# Autodesk Inventor assembly: czlon 1 i 2
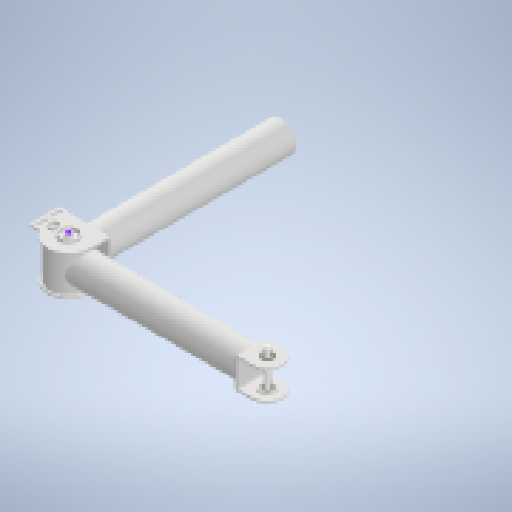
[picture p0: Inventor's stored thumbnail of the model, 512x512]
Saved by Autodesk Inventor 2023 (Build 270158000, 158)
## iProperties
Created: 2023-04-09
Part Number: czlon 1 i 2
Document SubType Name: Assembly
Designer: Wiktor
Author: Wiktor
## Documents named in this file (9)
- C:\Users\krzys\Documents\GitHub\Manipulator-Inventor\czlon 1 i 2.iam
- C:\Users\krzys\Documents\GitHub\Manipulator-Inventor\czlon i przekladnia.iam
- C:\Users\krzys\Documents\GitHub\Manipulator-Inventor\czlon 1 i 2\Design Accelerator\Łożysko1.iam
- C:\Users\krzys\Documents\GitHub\Manipulator-Inventor\Wał1.ipt
- C:\Users\krzys\Documents\GitHub\Manipulator-Inventor\czlon 1 i 2\Design Accelerator\Przekładnie walcowe1.iam
- C:\Users\krzys\Documents\GitHub\Manipulator-Inventor\czlon 1 i 2\Design Accelerator\Połączenie wpustowe1.iam
- C:\Users\krzys\Documents\GitHub\Manipulator-Inventor\czlon 2.ipt
- C:\Users\krzys\Documents\GitHub\Manipulator-Inventor\czlon 1 i 2\Design Accelerator\Łożysko2.iam
- C:\Users\krzys\Documents\GitHub\Manipulator-Inventor\Wał3.ipt
## Components (10 placed, 6 different names)
1. czlon i przekladnia:1 [sub-assembly] — Zestawiające:1, Zestawiające:2, Zestawiające:3, Zestawiające:4, Zestawiające:5, Kątowe:1, Równoległe:1
2. Łożysko:1 [sub-assembly] — Zestawiające:1, Zestawiające:2, Zestawiające:6, Zestawiające:7
3. Łożysko:3 [sub-assembly] — Zestawiające:3, Zestawiające:4, Zestawiające:5
4. Wał:1 — Zestawiające:6, Zestawiające:7, Kątowe:1, Zestawiające:10, Wstawiające:1
5. Przekładnie walcowe:1 [sub-assembly] — Wstawiające:1
6. Połączenie wpustowe:1 [sub-assembly]
7. czlon 2:1 — Zestawiające:10, Równoległe:1, Wstawiające:2, Wstawiające:3
8. Łożysko:4 [sub-assembly] — Wstawiające:3, Zestawiające:11, Równoległe:2, Kątowe:2
9. Łożysko:5 [sub-assembly] — Wstawiające:2
10. Wał:1 — Zestawiające:11, Równoległe:2, Kątowe:2
## Relationships (16: Mate 9, Insert 3, Angle 2, Flush 2)
- Zestawiające:1 [Mate]: czlon i przekladnia:1 ↔ Łożysko:1
- Zestawiające:2 [Mate]: czlon i przekladnia:1 ↔ Łożysko:1
- Zestawiające:3 [Mate]: czlon i przekladnia:1 ↔ Łożysko:3
- Zestawiające:4 [Mate]: czlon i przekladnia:1 ↔ Łożysko:3
- Zestawiające:5 [Mate]: czlon i przekladnia:1 ↔ Łożysko:3
- Zestawiające:6 [Mate]: Łożysko:1 ↔ Wał:1
- Zestawiające:7 [Mate]: Łożysko:1 ↔ Wał:1
- Kątowe:1 [Angle] (0 deg): czlon i przekladnia:1 ↔ Wał:1
- Zestawiające:10 [Mate]: Wał:1 ↔ czlon 2:1
- Równoległe:1 [Flush]: czlon i przekladnia:1 ↔ czlon 2:1
- Wstawiające:1 [Insert] (-20 mm): Wał:1 ↔ Przekładnie walcowe:1
- Wstawiające:2 [Insert]: czlon 2:1 ↔ Łożysko:5
- Wstawiające:3 [Insert]: czlon 2:1 ↔ Łożysko:4
- Zestawiające:11 [Mate]: Łożysko:4 ↔ Wał:1
- Równoległe:2 [Flush]: Łożysko:4 ↔ Wał:1
- Kątowe:2 [Angle] (0 deg): Łożysko:4 ↔ Wał:1
